# Autodesk Inventor assembly: 装配体
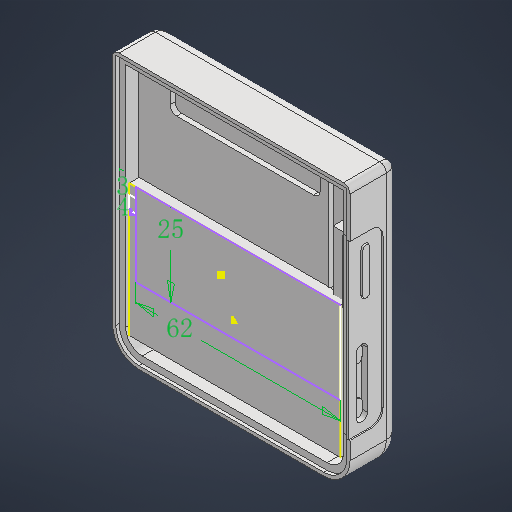
[picture p0: Inventor's stored thumbnail of the model, 512x512]
Saved by Autodesk Inventor 2025 (Build 290162000, 162)
## iProperties
Created: 2025-10-27
Part Number: 装配体
Document SubType Name: Assembly
Designer: XH
Author: XH
## Documents named in this file (8)
- D:\三星\装配体.iam
- D:\三星\键盘外壳.ipt
- D:\三星\电子\摄像头电路部分.ipt
- D:\三星\电子\上板电池.ipt
- D:\三星\电子\屏幕.ipt
- D:\三星\第二层板.ipt
- D:\三星\电子\大电池包裹.ipt
- D:\三星\dlc.iam
## Components (7 placed, 7 different names)
1. 键盘外壳:1 — 配合:16, 配合:17, 配合:18, 配合:19, 配合:21, 配合:22, 表面齐平:4
2. 摄像头电路部分:1 — 配合:1, 配合:10, 配合:13, 表面齐平:3
3. 上板电池:1 — 配合:1, 配合:20, 表面齐平:3
4. 屏幕:1 — 配合:10, 配合:18, 配合:19
5. 第二层板:1 — 配合:13, 配合:20
6. 大电池包裹:1 — 配合:16, 配合:17
7. dlc:1 [sub-assembly] — 配合:21, 配合:22, 表面齐平:4
## Relationships (12: Mate 10, Flush 2)
- 配合:1 [Mate] (2 mm): 摄像头电路部分:1 ↔ 上板电池:1
- 配合:20 [Mate]: 上板电池:1 ↔ 第二层板:1
- 配合:10 [Mate] (0.1 mm): 摄像头电路部分:1 ↔ 屏幕:1
- 配合:13 [Mate]: 摄像头电路部分:1 ↔ 第二层板:1
- 配合:16 [Mate]: 键盘外壳:1 ↔ 大电池包裹:1
- 配合:17 [Mate]: 键盘外壳:1 ↔ 大电池包裹:1
- 配合:18 [Mate]: 键盘外壳:1 ↔ 屏幕:1
- 配合:19 [Mate]: 键盘外壳:1 ↔ 屏幕:1
- 表面齐平:3 [Flush] (-6 mm): 摄像头电路部分:1 ↔ 上板电池:1
- 配合:21 [Mate]: 键盘外壳:1 ↔ dlc:1
- 配合:22 [Mate]: 键盘外壳:1 ↔ dlc:1
- 表面齐平:4 [Flush]: 键盘外壳:1 ↔ dlc:1
